# Autodesk Inventor assembly: Finished Tutorial
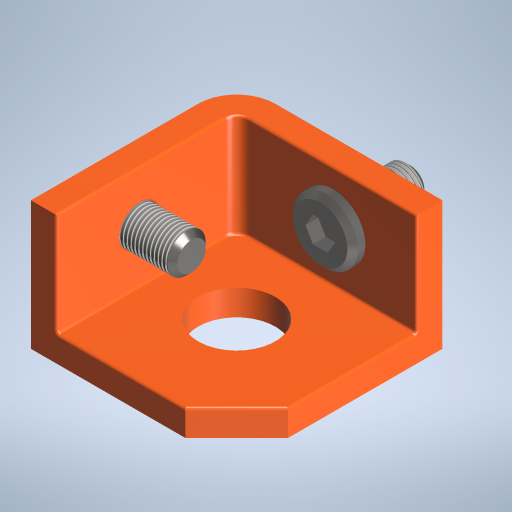
[picture p0: Inventor's stored thumbnail of the model, 512x512]
Saved by Autodesk Inventor 2024.4 (Build 284460000, 460)
## iProperties
Created: 2026-06-11
Part Number: Finished Tutorial
Document SubType Name: Assembly
Designer: stanc
Author: stanc
## Documents named in this file (3)
- C:\Users\stanc\OneDrive\Documents\GitHub\2026-2027-DesignTraining\Ivo\Finished Tutorial.iam
- C:\Users\stanc\OneDrive\Documents\GitHub\2026-2027-DesignTraining\Ivo\Tutorial Pt.1.ipt
- C:\Users\stanc\OneDrive\Documents\GitHub\2026-2027-DesignTraining\Ivo\Tutorial Pt.2.ipt
## Components (3 placed, 2 different names)
1. Tutorial Pt.1:1 — Mate:1, Mate:2, Angle:1, Mate:3, Mate:4, Angle:2
2. Tutorial Pt.2:1 — Mate:1, Mate:2, Angle:1
3. Tutorial Pt.2:2 — Mate:3, Mate:4, Angle:2
## Relationships (6: Mate 4, Angle 2)
- Mate:1: Tutorial Pt.1:1 ↔ Tutorial Pt.2:1
- Mate:2: Tutorial Pt.1:1 ↔ Tutorial Pt.2:1
- Angle:1 (0 deg): Tutorial Pt.1:1 ↔ Tutorial Pt.2:1
- Mate:3: Tutorial Pt.1:1 ↔ Tutorial Pt.2:2
- Mate:4: Tutorial Pt.1:1 ↔ Tutorial Pt.2:2
- Angle:2 (0 deg): Tutorial Pt.1:1 ↔ Tutorial Pt.2:2
